# Autodesk Inventor assembly: Crank_Slider_Fixer
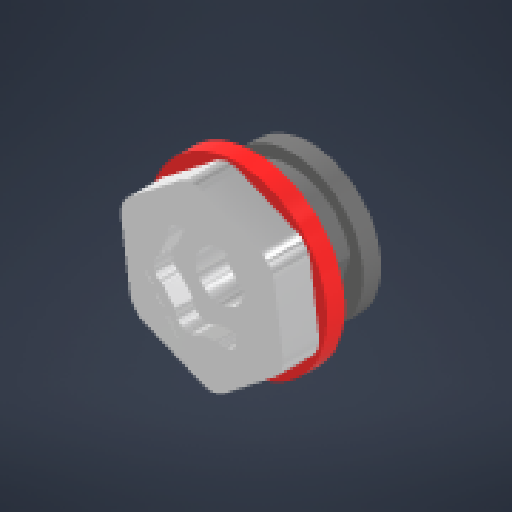
[picture p0: Inventor's stored thumbnail of the model, 512x512]
Saved by Autodesk Inventor 2024.3 (Build 283343000, 343)
## iProperties
Created: 2024-01-28
Part Number: Crank_Slider_Fixer
Document SubType Name: Assembly
Designer: 김대겸
Author: 김대겸
## Documents named in this file (5)
- C:\Users\ASUS\Desktop\ABD_2024_Eindhoven\MISUMI\Crank_Slider_Fixer.iam
- C:\Users\ASUS\Desktop\ABD_2024_Eindhoven\MISUMI\LED-0606.ipt
- C:\Users\ASUS\Desktop\ABD_2024_Eindhoven\v2_Frame\Ubber_Washer_1.5mm.ipt
- C:\Users\ASUS\Desktop\ABD_2024_Eindhoven\v2_Frame\Handmade tiered cover_9mm_Wide_ALU.ipt
- C:\Users\ASUS\Desktop\221006388707_3D\K1148.103\K1148.103\K1148.103.ipt
## Components (4 placed, 4 different names)
1. LED-0606:1 — 메이트:6, 메이트:7
2. Ubber_Washer_1.5mm:1 — 메이트:6, 메이트:7, 삽입:2
3. Handmade tiered cover_9mm_Wide_ALU:2 — 삽입:2, 삽입:3
4. K1148.103:1 — 삽입:3
## Relationships (4: Mate 2, Insert 2)
- 메이트:6 [Mate] (3 mm): LED-0606:1 ↔ Ubber_Washer_1.5mm:1
- 메이트:7 [Mate]: LED-0606:1 ↔ Ubber_Washer_1.5mm:1
- 삽입:2 [Insert]: Ubber_Washer_1.5mm:1 ↔ Handmade tiered cover_9mm_Wide_ALU:2
- 삽입:3 [Insert]: Handmade tiered cover_9mm_Wide_ALU:2 ↔ K1148.103:1
